# Autodesk Inventor assembly: 조립품1
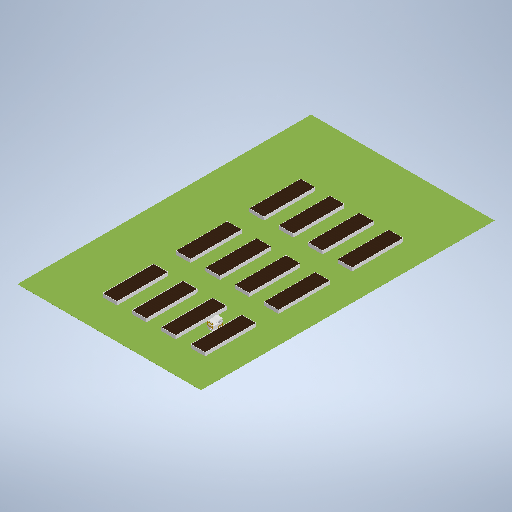
[picture p0: Inventor's stored thumbnail of the model, 512x512]
Saved by Autodesk Inventor 2025 (Build 290162010, 162A)
## iProperties
Created: 2024-06-18
Part Number: 조립품1
Document SubType Name: Assembly
Designer: user
Author: user
## Documents named in this file (5)
- J:\KWU_study_HW\roprog\Tomato-Is-All-You-Need\model_fusion\world\조립품1.iam
- J:\KWU_study_HW\roprog\Tomato-Is-All-You-Need\model_fusion\world\base.ipt
- J:\Inventor Files\model_fusion\조립품1.iam
- J:\KWU_study_HW\roprog\Tomato-Is-All-You-Need\model_fusion\world\farm pot.ipt
- J:\KWU_study_HW\roprog\Tomato-Is-All-You-Need\model_fusion\world\dirt.ipt
## Components (6 placed, 4 different names)
1. base:1
2. 조립품1:1 [sub-assembly]
3. farm pot:1 — 강체:1, 강체:2, 강체:3
4. dirt:1 — 강체:1
5. dirt:2 — 강체:3
6. dirt:3 — 강체:2
## Relationships (3: WeldJoint 3)
- 강체:1 [WeldJoint]: farm pot:1 ↔ dirt:1
- 강체:2 [WeldJoint]: farm pot:1 ↔ dirt:3
- 강체:3 [WeldJoint]: farm pot:1 ↔ dirt:2
